# Autodesk Inventor assembly: subsystem_3
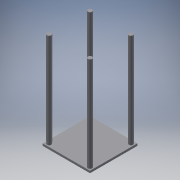
[picture p0: Inventor's stored thumbnail of the model, 180x180]
Saved by Autodesk Inventor 2019 (Build 230136000, 136)
## iProperties
Created: 2020-02-29
Part Number: subsystem_3
Document SubType Name: Assembly
Designer: Jayadev
Author: Jayadev
## Documents named in this file (3)
- G:\Inventor 2019\subsystem_3.iam
- G:\Inventor 2019\subsystem_3_rods.ipt
- G:\Inventor 2019\subsystem_3_base.ipt
## Components (5 placed, 2 different names)
1. subsystem_3_rods:1 — Mate:4, Flush:1
2. subsystem_3_rods:2 — Mate:3, Flush:2
3. subsystem_3_rods:3 — Mate:2, Flush:3
4. subsystem_3_rods:4 — Mate:1, Flush:4
5. subsystem_3_base:1 — Mate:1, Mate:2, Mate:3, Mate:4, Flush:1, Flush:2, Flush:3, Flush:4
## Relationships (8: Mate 4, Flush 4)
- Mate:1: subsystem_3_rods:4 ↔ subsystem_3_base:1
- Mate:2: subsystem_3_rods:3 ↔ subsystem_3_base:1
- Mate:3: subsystem_3_rods:2 ↔ subsystem_3_base:1
- Mate:4: subsystem_3_rods:1 ↔ subsystem_3_base:1
- Flush:1: subsystem_3_rods:1 ↔ subsystem_3_base:1
- Flush:2: subsystem_3_rods:2 ↔ subsystem_3_base:1
- Flush:3: subsystem_3_rods:3 ↔ subsystem_3_base:1
- Flush:4: subsystem_3_rods:4 ↔ subsystem_3_base:1
